# Autodesk Inventor assembly: s-assy-unit-j2
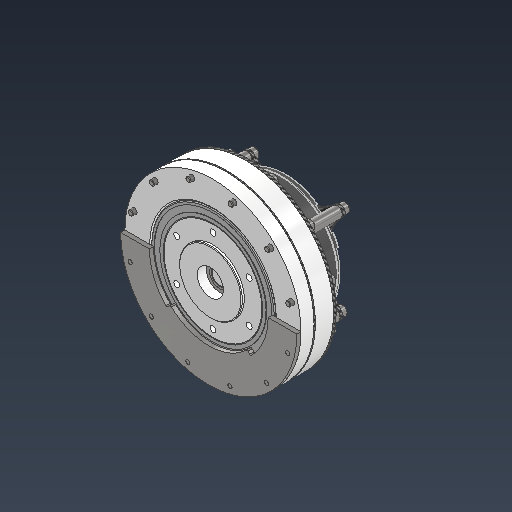
[picture p0: Inventor's stored thumbnail of the model, 512x512]
Saved by Autodesk Inventor 2021 (Build 250183000, 183)
## iProperties
Created: 2021-07-12
Part Number: s-assy-unit-j2
Document SubType Name: Assembly
Designer: yuta0
Mass: 876.37 g
Surface Area: 2474.15 cm^2
Volume: 379.417 cm^3
Density: 2.30978 g/cm^3
Author: yuta0
## Documents named in this file (5)
- C:\Users\yuta0\Desktop\catchrobo_robot\s-assy-unit-j2.iam
- C:\Users\yuta0\Desktop\catchrobo_robot\s-assy-sun_gear.iam
- C:\Users\yuta0\Desktop\catchrobo_robot\s-assy-unit-j2-2-gear.iam
- C:\Users\yuta0\Desktop\catchrobo_robot\s-assy-ring_gear.iam
- C:\Users\yuta0\Desktop\catchrobo_robot\steel_plate2.ipt
## Components (4 placed, 4 different names)
1. s-assy-sun_gear:1 [sub-assembly] — メイト:1, メイト:2
2. s-assy-unit-j2-2-gear:1 [sub-assembly] — メイト:1, フラッシュ:1, メイト:2, メイト:52, メイト:53
3. s-assy-ring_gear:1 [sub-assembly] — メイト:52, メイト:53, メイト:54, メイト:56
4. steel_plate2:1 — メイト:54, メイト:55, メイト:56
## Relationships (8: Mate 7, Flush 1)
- メイト:1 [Mate]: s-assy-sun_gear:1 ↔ s-assy-unit-j2-2-gear:1
- フラッシュ:1 [Flush]: s-assy-unit-j2-2-gear:1
- メイト:2 [Mate]: s-assy-sun_gear:1 ↔ s-assy-unit-j2-2-gear:1
- メイト:52 [Mate]: s-assy-unit-j2-2-gear:1 ↔ s-assy-ring_gear:1
- メイト:53 [Mate]: s-assy-unit-j2-2-gear:1 ↔ s-assy-ring_gear:1
- メイト:54 [Mate]: s-assy-ring_gear:1 ↔ steel_plate2:1
- メイト:55 [Mate]: steel_plate2:1
- メイト:56 [Mate]: s-assy-ring_gear:1 ↔ steel_plate2:1
